# Autodesk Inventor assembly: Ensamblaje5
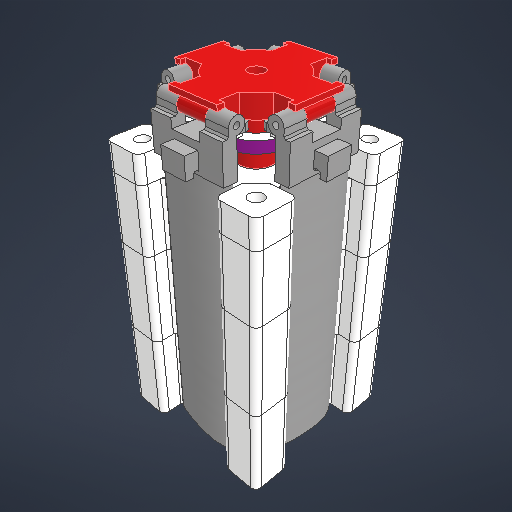
[picture p0: Inventor's stored thumbnail of the model, 512x512]
Saved by Autodesk Inventor 2026.1 (Build 301233000, 233)
## iProperties
Created: 2025-11-12
Part Number: Ensamblaje5
Document SubType Name: Assembly
Designer: usuario
Mass: 926.641 g
Surface Area: 2833.49 cm^2
Volume: 714.155 cm^3
Density: 1.29753 g/cm^3
Author: usuario
## Documents named in this file (14)
- C:\Users\vickh\Documents\Proyectos\Cansat_Huitzilin\3D\NuevoDiseno\Ensamblaje5.iam
- C:\Users\vickh\Documents\Proyectos\Cansat_Huitzilin\3D\NuevoDiseno\SujeccionHelices.ipt
- C:\Users\vickh\Documents\Proyectos\Cansat_Huitzilin\3D\NuevoDiseno\SistemLiberacion1.ipt
- C:\Users\vickh\Documents\Proyectos\Cansat_Huitzilin\3D\ViejoDiseno\Pieza9.ipt
- C:\Users\vickh\Documents\Proyectos\Cansat_Huitzilin\3D\NuevoDiseno\SistemaLiberacion2.2.ipt
- C:\Users\vickh\Documents\Proyectos\Cansat_Huitzilin\3D\NuevoDiseno\Electronica.ipt
- C:\Users\vickh\Documents\Proyectos\Cansat_Huitzilin\3D\NuevoDiseno\SemillasyAgua.ipt
- C:\Users\vickh\Documents\Proyectos\Cansat_Huitzilin\3D\NuevoDiseno\Huevo.ipt
- C:\Users\vickh\Documents\Proyectos\Cansat_Huitzilin\3D\NuevoDiseno\Ensamblaje5\AIP\FEA\f8yce27ts.fins
- C:\Users\vickh\Documents\Proyectos\Cansat_Huitzilin\3D\NuevoDiseno\Ensamblaje5\AIP\FEA\f8yce27ts.fsat
- C:\Users\vickh\Documents\Proyectos\Cansat_Huitzilin\3D\NuevoDiseno\Ensamblaje5\AIP\FEA\f8yce27ts.ftes
- C:\Users\vickh\Documents\Proyectos\Cansat_Huitzilin\3D\NuevoDiseno\Ensamblaje5\AIP\FEA\f8yce27ts.fwiz
- C:\Users\vickh\Documents\Proyectos\Cansat_Huitzilin\3D\NuevoDiseno\Ensamblaje5\AIP\FEA\f8yce27vk.fmsh
- C:\Users\vickh\Documents\Proyectos\Cansat_Huitzilin\3D\NuevoDiseno\Ensamblaje5\AIP\FEA\f8yce27vl.fres
## Components (10 placed, 7 different names)
1. SujeccionHelices:1 — Cilíndrica:1, Insertar:1, De rotación:1, De rotación:2, De rotación:3, De rotación:4
2. SistemLiberacion1:1 — Cilíndrica:1
3. Pieza9:1 — De rotación:4
4. Pieza9:2 — De rotación:2
5. Pieza9:3 — De rotación:1
6. Pieza9:4 — De rotación:3
7. SistemaLiberacion2.2:1 — Insertar:1, Coincidencia:1, Nivelación:1, Nivelación:2, Coincidencia:4
8. Electronica:1 — Coincidencia:1, Nivelación:1, Nivelación:2, Coincidencia:4, Coincidencia:5, Nivelación:3, Nivelación:4
9. SemillasyAgua:1 — Coincidencia:6, Nivelación:5, Nivelación:6
10. Huevo:1 — Coincidencia:5, Nivelación:3, Nivelación:4, Coincidencia:6, Nivelación:5, Nivelación:6
## Relationships (16: Flush 6, RevoluteJoint 4, Mate 4, CylindricalJoint 1, Insert 1)
- Cilíndrica:1 [CylindricalJoint]: SujeccionHelices:1 ↔ SistemLiberacion1:1
- Insertar:1: SujeccionHelices:1 ↔ SistemaLiberacion2.2:1
- De rotación:1 [RevoluteJoint]: SujeccionHelices:1 ↔ Pieza9:3
- De rotación:2 [RevoluteJoint]: SujeccionHelices:1 ↔ Pieza9:2
- De rotación:3 [RevoluteJoint]: SujeccionHelices:1 ↔ Pieza9:4
- De rotación:4 [RevoluteJoint]: SujeccionHelices:1 ↔ Pieza9:1
- Coincidencia:1 [Mate]: SistemaLiberacion2.2:1 ↔ Electronica:1
- Nivelación:1 [Flush]: SistemaLiberacion2.2:1 ↔ Electronica:1
- Nivelación:2 [Flush]: SistemaLiberacion2.2:1 ↔ Electronica:1
- Coincidencia:4 [Mate]: SistemaLiberacion2.2:1 ↔ Electronica:1
- Coincidencia:5 [Mate]: Electronica:1 ↔ Huevo:1
- Nivelación:3 [Flush]: Electronica:1 ↔ Huevo:1
- Nivelación:4 [Flush]: Electronica:1 ↔ Huevo:1
- Coincidencia:6 [Mate]: SemillasyAgua:1 ↔ Huevo:1
- Nivelación:5 [Flush]: SemillasyAgua:1 ↔ Huevo:1
- Nivelación:6 [Flush]: SemillasyAgua:1 ↔ Huevo:1
## Named parameters: sa_0 = 0, sa_1 = -981, sa_2 = 0, sa_3 = 1.5e+06
note: some values were not read from the file. Shown as the stored number, unit unknown: "sa_0", "sa_1", "sa_2", "sa_3".
